# Autodesk Inventor assembly: CE-7.1.1_CE-2.1.4_PZ
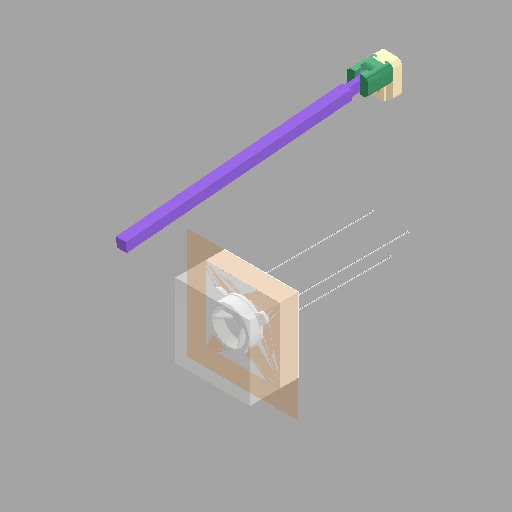
[picture p0: Inventor's stored thumbnail of the model, 512x512]
Saved by Autodesk Inventor 2024 (Build 280153000, 153)
## iProperties
Created: 2024-02-25
Part Number: CE-7.1.1_CE-2.1.4_PZ
Document SubType Name: Assembly
Designer: Alex
Author: Alex
## Documents named in this file (11)
- C:\Shared\alex-bartella-schoolwork\4z03\Week 6\CE-7.1.1_CE-2.1.4_PZ.iam
- C:\Shared\alex-bartella-schoolwork\4z03\Week 6\CE-7.1.1_CE-2.1.4_MP.ipt
- C:\Shared\alex-bartella-schoolwork\4z03\Week 6\CE-7.1.1_CE-2.1.4_WP.ipt
- C:\Shared\alex-bartella-schoolwork\4z03\Week 6\CE-7.1.1_CE-2.1.4_CR_Base.ipt
- C:\Shared\alex-bartella-schoolwork\4z03\Week 6\CE-7.1.1_CE-2.1.4_CR_1.ipt
- C:\Shared\alex-bartella-schoolwork\4z03\Week 6\CE-7.1.1_CE-2.1.4_CV_Base.ipt
- C:\Shared\alex-bartella-schoolwork\4z03\Week 6\CE-7.1.1_CE-2.1.4_CV_1.ipt
- C:\Shared\alex-bartella-schoolwork\4z03\Week 6\Lifters\DME_Flat Core Blades 1\CE-7.1.1_CE-2.1.4_LA1.iam
- C:\Shared\alex-bartella-schoolwork\4z03\Week 6\Ejectors\DME_AH\EP Group1.0\CE-7.1.1_CE-2.1.4_EP Group1_EP4.ipt
- C:\Shared\alex-bartella-schoolwork\4z03\Week 6\Ejectors\DME_AH\EP Group1.0\CE-7.1.1_CE-2.1.4_EP Group1_EP5.ipt
- C:\Shared\alex-bartella-schoolwork\4z03\Week 6\Ejectors\DME_AH\EP Group1.0\CE-7.1.1_CE-2.1.4_EP Group1_EP6.ipt
## Components (10 placed, 10 different names)
1. CE-7.1.1_CE-2.1.4_MP:1 — Flush:1, Flush:2, Flush:3, Flush:4, Flush:5, Flush:6, Flush:23
2. CE-7.1.1_CE-2.1.4_WP:1 — Flush:4, Flush:5, Flush:6
3. CE-7.1.1_CE-2.1.4_CR_Base:1 — Flush:7, Flush:8, Flush:9, Flush:13, Flush:14, Flush:15
4. CE-7.1.1_CE-2.1.4_CR_1:1 — Flush:13, Flush:14, Flush:15
5. CE-7.1.1_CE-2.1.4_CV_Base:1 — Flush:10, Flush:11, Flush:12, Flush:16, Flush:17, Flush:18
6. CE-7.1.1_CE-2.1.4_CV_1:1 — Flush:16, Flush:17, Flush:18
7. CE-7.1.1_CE-2.1:1 [sub-assembly]
8. CE-7.1.1_CE-2.1.4_EP Group1_EP4:1 — Mate:1, Flush:20, Angle:1, Flush:23
9. CE-7.1.1_CE-2.1.4_EP Group1_EP5:1 — Mate:2, Flush:21, Angle:2
10. CE-7.1.1_CE-2.1.4_EP Group1_EP6:1 — Mate:3, Flush:22, Angle:3
## Relationships (28: Flush 22, Mate 3, Angle 3)
- Flush:1: CE-7.1.1_CE-2.1.4_MP:1
- Flush:2: CE-7.1.1_CE-2.1.4_MP:1
- Flush:3: CE-7.1.1_CE-2.1.4_MP:1
- Flush:4: CE-7.1.1_CE-2.1.4_MP:1 ↔ CE-7.1.1_CE-2.1.4_WP:1
- Flush:5: CE-7.1.1_CE-2.1.4_MP:1 ↔ CE-7.1.1_CE-2.1.4_WP:1
- Flush:6: CE-7.1.1_CE-2.1.4_MP:1 ↔ CE-7.1.1_CE-2.1.4_WP:1
- Flush:7: CE-7.1.1_CE-2.1.4_CR_Base:1
- Flush:8: CE-7.1.1_CE-2.1.4_CR_Base:1
- Flush:9: CE-7.1.1_CE-2.1.4_CR_Base:1
- Flush:10: CE-7.1.1_CE-2.1.4_CV_Base:1
- Flush:11: CE-7.1.1_CE-2.1.4_CV_Base:1
- Flush:12: CE-7.1.1_CE-2.1.4_CV_Base:1
- Flush:13: CE-7.1.1_CE-2.1.4_CR_Base:1 ↔ CE-7.1.1_CE-2.1.4_CR_1:1
- Flush:14: CE-7.1.1_CE-2.1.4_CR_Base:1 ↔ CE-7.1.1_CE-2.1.4_CR_1:1
- Flush:15: CE-7.1.1_CE-2.1.4_CR_Base:1 ↔ CE-7.1.1_CE-2.1.4_CR_1:1
- Flush:16: CE-7.1.1_CE-2.1.4_CV_Base:1 ↔ CE-7.1.1_CE-2.1.4_CV_1:1
- Flush:17: CE-7.1.1_CE-2.1.4_CV_Base:1 ↔ CE-7.1.1_CE-2.1.4_CV_1:1
- Flush:18: CE-7.1.1_CE-2.1.4_CV_Base:1 ↔ CE-7.1.1_CE-2.1.4_CV_1:1
- Mate:1: CE-7.1.1_CE-2.1.4_EP Group1_EP4:1
- Flush:20: CE-7.1.1_CE-2.1.4_EP Group1_EP4:1
- Angle:1 (180 deg): CE-7.1.1_CE-2.1.4_EP Group1_EP4:1
- Mate:2: CE-7.1.1_CE-2.1.4_EP Group1_EP5:1
- Flush:21: CE-7.1.1_CE-2.1.4_EP Group1_EP5:1
- Angle:2 (180 deg): CE-7.1.1_CE-2.1.4_EP Group1_EP5:1
- Mate:3: CE-7.1.1_CE-2.1.4_EP Group1_EP6:1
- Flush:22: CE-7.1.1_CE-2.1.4_EP Group1_EP6:1
- Angle:3 (180 deg): CE-7.1.1_CE-2.1.4_EP Group1_EP6:1
- Flush:23: CE-7.1.1_CE-2.1.4_MP:1 ↔ CE-7.1.1_CE-2.1.4_EP Group1_EP4:1
